# Autodesk Inventor assembly: BOX
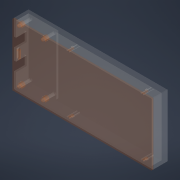
[picture p0: Inventor's stored thumbnail of the model, 180x180]
Saved by Autodesk Inventor 2022 (Build 260153000, 153)
## iProperties
Created: 2022-10-04
Part Number: BOX
Document SubType Name: Assembly
Designer: 15628
Author: 15628
## Documents named in this file (3)
- C:\Users\15628\Desktop\BATTERY\BOX.iam
- C:\Users\15628\Desktop\BATTERY\BOT.ipt
- C:\Users\15628\Desktop\BATTERY\TOP.ipt
## Components (2 placed, 2 different names)
1. BOT:1 — 插入:1
2. TOP:1 — 插入:1
## Relationships (1: Insert 1)
- 插入:1 [Insert] (-4.3 mm): BOT:1 ↔ TOP:1
